# Autodesk Inventor assembly: Pancake_Switch Lever Assy
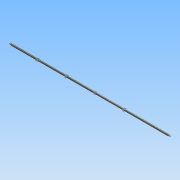
[picture p0: Inventor's stored thumbnail of the model, 180x180]
Saved by Autodesk Inventor 2018.1 (Build 221171000, 171)
## iProperties
Created: 2019-03-01
Part Number: Pancake_Switch Lever Assy
Document SubType Name: Assembly
Designer: James
Author: James
## Documents named in this file (3)
- C:\Users\admin\Desktop\Ball Sorting Machine\Ball-Sorting-Machine\Pancake Sort\Pancake_Switch Lever Assy.iam
- C:\Users\admin\Desktop\Ball Sorting Machine\Ball-Sorting-Machine\Pancake Sort\Pancake_Switch Lever Shaft.ipt
- C:\Users\admin\Desktop\Ball Sorting Machine\Ball-Sorting-Machine\Pancake Sort\BS 3673 - 6mm External Circlip.ipt
## Components (9 placed, 2 different names)
1. Pancake_Switch Lever Shaft:1 — Flush:1, Flush:2, Flush:3, Mate:1, Mate:2, Mate:3, Mate:4
2. BS 3673 - 6mm External Circlip:1 — Mate:1, Mate:4, Flush:4, Angle:1
3. BS 3673 - 6mm External Circlip:2 — Mate:2, Mate:3, Flush:4
4. BS 3673 - 6mm External Circlip:3
5. BS 3673 - 6mm External Circlip:4
6. BS 3673 - 6mm External Circlip:5
7. BS 3673 - 6mm External Circlip:6
8. BS 3673 - 6mm External Circlip:7
9. BS 3673 - 6mm External Circlip:8
## Component patterns: (4 elements, first: BS 3673 - 6mm External Circlip:1 + BS 3673 - 6mm External Circlip:2)
## Relationships (9: Flush 4, Mate 4, Angle 1)
- Flush:1: Pancake_Switch Lever Shaft:1
- Flush:2: Pancake_Switch Lever Shaft:1
- Flush:3: Pancake_Switch Lever Shaft:1
- Mate:1: Pancake_Switch Lever Shaft:1 ↔ BS 3673 - 6mm External Circlip:1
- Mate:2: Pancake_Switch Lever Shaft:1 ↔ BS 3673 - 6mm External Circlip:2
- Mate:3: Pancake_Switch Lever Shaft:1 ↔ BS 3673 - 6mm External Circlip:2
- Mate:4: Pancake_Switch Lever Shaft:1 ↔ BS 3673 - 6mm External Circlip:1
- Flush:4: BS 3673 - 6mm External Circlip:1 ↔ BS 3673 - 6mm External Circlip:2
- Angle:1 (0 deg): BS 3673 - 6mm External Circlip:1
